# Autodesk Inventor assembly: Everything
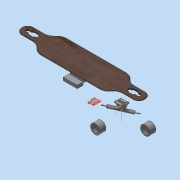
[picture p0: Inventor's stored thumbnail of the model, 180x180]
Saved by Autodesk Inventor 2017 (Build 210142000, 142)
## iProperties
Created: 2016-01-09
Part Number: Everything
Document SubType Name: Assembly
Designer: JoshuaYuan
Author: JoshuaYuan
## Documents named in this file (8)
- C:\Other Project Stuff\Longboard\Everything.iam
- C:\Other Project Stuff\Longboard\arduino_uno.ipt
- C:\Other Project Stuff\Longboard\battery.ipt
- C:\Other Project Stuff\Longboard\Wheels.ipt
- C:\Other Project Stuff\Longboard\bearing_ABEC_7.ipt
- C:\Other Project Stuff\Longboard\50cal_truck.ipt
- C:\Other Project Stuff\Longboard\50cal_baseplate.ipt
- C:\Other Project Stuff\Longboard\Deck.ipt
## Components (13 placed, 7 different names)
1. arduino_uno:1
2. battery:1
3. battery:2
4. Wheels:1
5. Wheels:2 — Insert:5, Insert:6
6. Wheels:3 — Insert:3, Insert:4
7. bearing_ABEC_7:3 — Insert:4
8. bearing_ABEC_7:4 — Insert:5
9. bearing_ABEC_7:5 — Insert:6
10. bearing_ABEC_7:6 — Insert:3
11. 50cal_truck:1 — Mate:1, Mate:2
12. 50cal_baseplate:1 — Mate:1, Mate:2
13. Deck:1
## Relationships (6: Insert 4, Mate 2)
- Insert:3: Wheels:3 ↔ bearing_ABEC_7:6
- Insert:4: Wheels:3 ↔ bearing_ABEC_7:3
- Insert:5: Wheels:2 ↔ bearing_ABEC_7:4
- Insert:6: Wheels:2 ↔ bearing_ABEC_7:5
- Mate:1: 50cal_truck:1 ↔ 50cal_baseplate:1
- Mate:2: 50cal_truck:1 ↔ 50cal_baseplate:1
